# Autodesk Inventor assembly: 1_2x1_2-hexBearingJoinedAandB
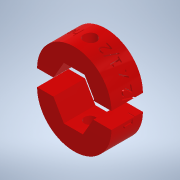
[picture p0: Inventor's stored thumbnail of the model, 180x180]
Saved by Autodesk Inventor 2022.1 (Build 261234000, 234)
## iProperties
Created: 2021-07-22
Part Number: 1_2x1_2-hexBearingJoinedAandB
Document SubType Name: Assembly
Designer: robst
Author: robst
## Documents named in this file (3)
- C:\git\CAD-Development\robSteele\ShapeWays\TelescopeProjects\TelescopeMountNov2020\1_2x1_2-hexBearingJoinedAandB.iam
- C:\git\CAD-Development\robSteele\ShapeWays\TelescopeProjects\TelescopeMountNov2020\1_2x1_2-hexBearingSplitA.ipt
- C:\git\CAD-Development\robSteele\ShapeWays\TelescopeProjects\TelescopeMountNov2020\1_2x1_2-hexBearingSplitB.ipt
## Components (2 placed, 2 different names)
1. 1_2x1_2-hexBearingSplitA:1 — Mate:1, Flush:1
2. 1_2x1_2-hexBearingSplitB:1 — Mate:1, Flush:1
## Relationships (2: Mate 1, Flush 1)
- Mate:1 (6.35 mm): 1_2x1_2-hexBearingSplitA:1 ↔ 1_2x1_2-hexBearingSplitB:1
- Flush:1: 1_2x1_2-hexBearingSplitA:1 ↔ 1_2x1_2-hexBearingSplitB:1
